# Autodesk Inventor assembly: Brazo Robótivo 2023 v144
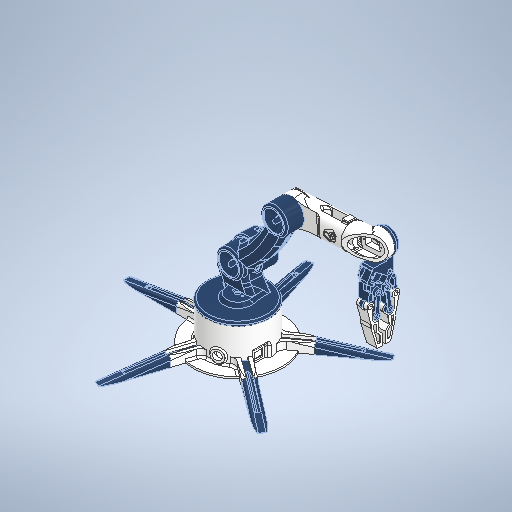
[picture p0: Inventor's stored thumbnail of the model, 512x512]
Saved by Autodesk Inventor 2025.2 (Build 292293000, 293)
## iProperties
Created: 2024-04-02
Part Number: Brazo Robótivo 2023 v144
Document SubType Name: Assembly
Designer: Gustavo Sousa
Sending System: Autodesk Translation Framework v12.20.1.177
Preprocessor: ST-DEVELOPER v20
Title: Brazo Robtivo 2023 v144.step
## Documents named in this file (22)
- C:\Users\lucas\OneDrive\Documentos\Documentos\Gustavo\Mozangao\Projeto Base (5140)\braco_robotico\Brazo Robótivo 2023 v144\Brazo Robótivo 2023 v144\Brazo Robótivo 2023 v144.iam
- C:\Users\lucas\OneDrive\Documentos\Documentos\Gustavo\Mozangao\Projeto Base (5140)\braco_robotico\Brazo Robótivo 2023 v144\Brazo Robótivo 2023 v144\Engranaje1.ipt
- C:\Users\lucas\OneDrive\Documentos\Documentos\Gustavo\Mozangao\Projeto Base (5140)\braco_robotico\Brazo Robótivo 2023 v144\Brazo Robótivo 2023 v144\Engranaje2.ipt
- C:\Users\lucas\OneDrive\Documentos\Documentos\Gustavo\Mozangao\Projeto Base (5140)\braco_robotico\Brazo Robótivo 2023 v144\Brazo Robótivo 2023 v144\Barra2.ipt
- C:\Users\lucas\OneDrive\Documentos\Documentos\Gustavo\Mozangao\Projeto Base (5140)\braco_robotico\Brazo Robótivo 2023 v144\Brazo Robótivo 2023 v144\Barra1.ipt
- C:\Users\lucas\OneDrive\Documentos\Documentos\Gustavo\Mozangao\Projeto Base (5140)\braco_robotico\Brazo Robótivo 2023 v144\Brazo Robótivo 2023 v144\Pinza1.ipt
- C:\Users\lucas\OneDrive\Documentos\Documentos\Gustavo\Mozangao\Projeto Base (5140)\braco_robotico\Brazo Robótivo 2023 v144\Brazo Robótivo 2023 v144\Pinza2.ipt
- C:\Users\lucas\OneDrive\Documentos\Documentos\Gustavo\Mozangao\Projeto Base (5140)\braco_robotico\Brazo Robótivo 2023 v144\Brazo Robótivo 2023 v144\Base de la garra.ipt
- C:\Users\lucas\OneDrive\Documentos\Documentos\Gustavo\Mozangao\Projeto Base (5140)\braco_robotico\Brazo Robótivo 2023 v144\Brazo Robótivo 2023 v144\Base (1) (1).ipt
- C:\Users\lucas\OneDrive\Documentos\Documentos\Gustavo\Mozangao\Projeto Base (5140)\braco_robotico\Brazo Robótivo 2023 v144\Brazo Robótivo 2023 v144\Antebrazo (4).ipt
- C:\Users\lucas\OneDrive\Documentos\Documentos\Gustavo\Mozangao\Projeto Base (5140)\braco_robotico\Brazo Robótivo 2023 v144\Brazo Robótivo 2023 v144\Muñeca.ipt
- C:\Users\lucas\OneDrive\Documentos\Documentos\Gustavo\Mozangao\Projeto Base (5140)\braco_robotico\Brazo Robótivo 2023 v144\Brazo Robótivo 2023 v144\Eje Central.ipt
- C:\Users\lucas\OneDrive\Documentos\Documentos\Gustavo\Mozangao\Projeto Base (5140)\braco_robotico\Brazo Robótivo 2023 v144\Brazo Robótivo 2023 v144\Tapa Eje.ipt
- C:\Users\lucas\OneDrive\Documentos\Documentos\Gustavo\Mozangao\Projeto Base (5140)\braco_robotico\Brazo Robótivo 2023 v144\Brazo Robótivo 2023 v144\Tapa Base.ipt
- C:\Users\lucas\OneDrive\Documentos\Documentos\Gustavo\Mozangao\Projeto Base (5140)\braco_robotico\Brazo Robótivo 2023 v144\Brazo Robótivo 2023 v144\Brazo.ipt
- C:\Users\lucas\OneDrive\Documentos\Documentos\Gustavo\Mozangao\Projeto Base (5140)\braco_robotico\Brazo Robótivo 2023 v144\Brazo Robótivo 2023 v144\Tapa garra.ipt
- C:\Users\lucas\OneDrive\Documentos\Documentos\Gustavo\Mozangao\Projeto Base (5140)\braco_robotico\Brazo Robótivo 2023 v144\Brazo Robótivo 2023 v144\Pata1.ipt
- C:\Users\lucas\OneDrive\Documentos\Documentos\Gustavo\Mozangao\Projeto Base (5140)\braco_robotico\Brazo Robótivo 2023 v144\Brazo Robótivo 2023 v144\Pata2.ipt
- C:\Users\lucas\OneDrive\Documentos\Documentos\Gustavo\Mozangao\Projeto Base (5140)\braco_robotico\Brazo Robótivo 2023 v144\Brazo Robótivo 2023 v144\Pata3.ipt
- C:\Users\lucas\OneDrive\Documentos\Documentos\Gustavo\Mozangao\Projeto Base (5140)\braco_robotico\Brazo Robótivo 2023 v144\Brazo Robótivo 2023 v144\Pata4.ipt
- C:\Users\lucas\OneDrive\Documentos\Documentos\Gustavo\Mozangao\Projeto Base (5140)\braco_robotico\Brazo Robótivo 2023 v144\Brazo Robótivo 2023 v144\Pata5.ipt
- C:\Users\lucas\OneDrive\Documentos\Documentos\Gustavo\Mozangao\Projeto Base (5140)\braco_robotico\Brazo Robótivo 2023 v144\Brazo Robótivo 2023 v144\Seguro de servomotor.ipt
## Components (21 placed, 21 different names)
1. Engranaje1:1 — Coincidente:24, Coincidente:25, Inserir:10
2. Engranaje2:1 — Coincidente:22, Coincidente:23, Inserir:11
3. Barra2:1 — Inserir:8, Coincidente:27
4. Barra1:1 — Inserir:9, Coincidente:26
5. Pinza1:1 — Inserir:10, Coincidente:26
6. Pinza2:1 — Inserir:11, Coincidente:27
7. Base de la garra:1 — Inserir:6, Coincidente:21, Inserir:8, Inserir:9, Inserir:12
8. Base (1) (1):1 — Coincidente:7, Coincidente:8, Coincidente:9, Coincidente:10, Coincidente:11, Coincidente:12, Coincidente:13, Coincidente:14, Coincidente:15, Coincidente:16, Coincidente:17, Coincidente:18, Alinhado:1, Alinhado:2, Alinhado:3, Inserir:1
9. Antebrazo (4):1 — Inserir:2, Inserir:4
10. Muñeca:1 — Inserir:5, Inserir:12
11. Eje Central:1 — Inserir:1, Coincidente:19, Coincidente:20, Inserir:2
12. Tapa Eje:1 — Coincidente:19, Coincidente:20
13. Tapa Base:1 — Coincidente:17, Coincidente:18
14. Brazo:1 — Inserir:3, Inserir:4, Inserir:5
15. Tapa garra:1 — Inserir:6, Coincidente:21, Coincidente:22, Coincidente:23, Coincidente:24, Coincidente:25
16. Pata1:1 — Coincidente:9, Coincidente:10
17. Pata2:1 — Coincidente:11, Coincidente:12
18. Pata3:1 — Coincidente:15, Coincidente:16
19. Pata4:1 — Coincidente:13, Coincidente:14
20. Pata5:1 — Coincidente:7, Coincidente:8
21. Seguro de servomotor:1 — Inserir:3
## Relationships (35: Mate 21, Insert 11, Flush 3)
- Coincidente:7 [Mate]: Base (1) (1):1 ↔ Pata5:1
- Coincidente:8 [Mate]: Base (1) (1):1 ↔ Pata5:1
- Coincidente:9 [Mate]: Base (1) (1):1 ↔ Pata1:1
- Coincidente:10 [Mate]: Base (1) (1):1 ↔ Pata1:1
- Coincidente:11 [Mate]: Base (1) (1):1 ↔ Pata2:1
- Coincidente:12 [Mate]: Base (1) (1):1 ↔ Pata2:1
- Coincidente:13 [Mate]: Base (1) (1):1 ↔ Pata4:1
- Coincidente:14 [Mate]: Base (1) (1):1 ↔ Pata4:1
- Coincidente:15 [Mate]: Base (1) (1):1 ↔ Pata3:1
- Coincidente:16 [Mate]: Base (1) (1):1 ↔ Pata3:1
- Coincidente:17 [Mate]: Base (1) (1):1 ↔ Tapa Base:1
- Coincidente:18 [Mate]: Base (1) (1):1 ↔ Tapa Base:1
- Alinhado:1 [Flush]: Base (1) (1):1
- Alinhado:2 [Flush]: Base (1) (1):1
- Alinhado:3 [Flush]: Base (1) (1):1
- Inserir:1: Base (1) (1):1 ↔ Eje Central:1
- Coincidente:19 [Mate]: Eje Central:1 ↔ Tapa Eje:1
- Coincidente:20 [Mate] (1.05 mm): Eje Central:1 ↔ Tapa Eje:1
- Inserir:2: Antebrazo (4):1 ↔ Eje Central:1
- Inserir:3: Brazo:1 ↔ Seguro de servomotor:1
- Inserir:4: Antebrazo (4):1 ↔ Brazo:1
- Inserir:5: Muñeca:1 ↔ Brazo:1
- Inserir:6: Base de la garra:1 ↔ Tapa garra:1
- Coincidente:21 [Mate]: Base de la garra:1 ↔ Tapa garra:1
- Inserir:8: Barra2:1 ↔ Base de la garra:1
- Inserir:9: Barra1:1 ↔ Base de la garra:1
- Coincidente:22 [Mate]: Engranaje2:1 ↔ Tapa garra:1
- Coincidente:23 [Mate]: Engranaje2:1 ↔ Tapa garra:1
- Coincidente:24 [Mate]: Engranaje1:1 ↔ Tapa garra:1
- Coincidente:25 [Mate]: Engranaje1:1 ↔ Tapa garra:1
- Inserir:10 (0.5 mm): Engranaje1:1 ↔ Pinza1:1
- Coincidente:26 [Mate]: Barra1:1 ↔ Pinza1:1
- Inserir:11: Engranaje2:1 ↔ Pinza2:1
- Coincidente:27 [Mate]: Barra2:1 ↔ Pinza2:1
- Inserir:12: Base de la garra:1 ↔ Muñeca:1
